# Autodesk Inventor assembly: use this - gimme that tech award
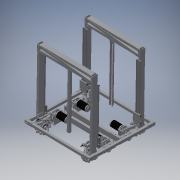
[picture p0: Inventor's stored thumbnail of the model, 180x180]
Saved by Autodesk Inventor 2018 (Build 220112000, 112)
## iProperties
Created: 2019-01-10
Part Number: use this - gimme that tech award
Document SubType Name: Assembly
Designer: maste
Author: maste
## Documents named in this file (6)
- C:\Users\s-2512711\Desktop\Github\2019CAD\Drivebase but Calvin is a mad man\use this - gimme that tech award.iam
- C:\Users\s-2512711\Desktop\Github\2019CAD\Drivebase but Calvin is a mad man\Slidey Mecanum L thing V2.iam
- C:\Users\s-2512711\Desktop\Github\2019CAD\Drivebase but Calvin is a mad man\WW_10_40_10_AL_2.ipt
- C:\Users\s-2512711\Desktop\Github\2019CAD\Drivebase but Calvin is a mad man\91292A197_TYPE 18-8 SS SOCKET HEAD CAP SCREW (1).ipt
- C:\Users\s-2512711\Desktop\Github\2019CAD\Drivebase but Calvin is a mad man\93625A200_TYPE 18-8 STAINLESS STL NYLON-INSERT LOCKNUT.ipt
- C:\Users\s-2512711\Desktop\Github\2019CAD\Drivebase but Calvin is a mad man\Bumper Frame.iam
## Components (23 placed, 5 different names)
1. Slidey Mecanum L thing V2:1 [sub-assembly] — Mate:59, Mate:60, Mate:61, Mate:62, Flush:5, Flush:6, Flush:7, Mate:118
2. Slidey Mecanum L thing V2:2 [sub-assembly] — Mate:55, Mate:56, Mate:57, Mate:58, Flush:3, Flush:4, Mate:115, Mate:116, Mate:117, Flush:7
3. WW_10_40_10_AL_2:1 — Mate:57, Mate:58, Flush:3, Mate:76, Mate:77, Mate:78, Mate:79
4. WW_10_40_10_AL_2:2 — Mate:59, Mate:60, Flush:5, Mate:88, Mate:89, Mate:90, Mate:91
5. WW_10_40_10_AL_2:3 — Mate:61, Mate:62, Flush:6, Mate:84, Mate:85, Mate:86, Mate:87
6. WW_10_40_10_AL_2:4 — Mate:55, Mate:56, Flush:4, Mate:80, Mate:81, Mate:82, Mate:83
7. 91292A197_TYPE 18-8 SS SOCKET HEAD CAP SCREW (1):1 — Mate:76, Mate:77, Mate:106
8. 91292A197_TYPE 18-8 SS SOCKET HEAD CAP SCREW (1):2 — Mate:78, Mate:79, Mate:107
9. 91292A197_TYPE 18-8 SS SOCKET HEAD CAP SCREW (1):3 — Mate:80, Mate:81, Mate:110
10. 91292A197_TYPE 18-8 SS SOCKET HEAD CAP SCREW (1):4 — Mate:82, Mate:83, Mate:111
11. 91292A197_TYPE 18-8 SS SOCKET HEAD CAP SCREW (1):5 — Mate:84, Mate:85, Mate:103
12. 91292A197_TYPE 18-8 SS SOCKET HEAD CAP SCREW (1):6 — Mate:86, Mate:87, Mate:102
13. 91292A197_TYPE 18-8 SS SOCKET HEAD CAP SCREW (1):7 — Mate:90, Mate:91, Mate:99
14. 91292A197_TYPE 18-8 SS SOCKET HEAD CAP SCREW (1):8 — Mate:88, Mate:89, Mate:98
15. 93625A200_TYPE 18-8 STAINLESS STL NYLON-INSERT LOCKNUT:1 — Mate:111
16. 93625A200_TYPE 18-8 STAINLESS STL NYLON-INSERT LOCKNUT:2 — Mate:110
17. 93625A200_TYPE 18-8 STAINLESS STL NYLON-INSERT LOCKNUT:3 — Mate:106
18. 93625A200_TYPE 18-8 STAINLESS STL NYLON-INSERT LOCKNUT:4 — Mate:107
19. 93625A200_TYPE 18-8 STAINLESS STL NYLON-INSERT LOCKNUT:6 — Mate:99
20. 93625A200_TYPE 18-8 STAINLESS STL NYLON-INSERT LOCKNUT:7 — Mate:98
21. 93625A200_TYPE 18-8 STAINLESS STL NYLON-INSERT LOCKNUT:8 — Mate:103
22. 93625A200_TYPE 18-8 STAINLESS STL NYLON-INSERT LOCKNUT:9 — Mate:102
23. Bumper Frame:1 [sub-assembly] — Mate:115, Mate:116, Mate:117, Mate:118
## Relationships (41: Mate 36, Flush 5)
- Mate:55: Slidey Mecanum L thing V2:2 ↔ WW_10_40_10_AL_2:4
- Mate:56: Slidey Mecanum L thing V2:2 ↔ WW_10_40_10_AL_2:4
- Mate:57: Slidey Mecanum L thing V2:2 ↔ WW_10_40_10_AL_2:1
- Mate:58: Slidey Mecanum L thing V2:2 ↔ WW_10_40_10_AL_2:1
- Mate:59: Slidey Mecanum L thing V2:1 ↔ WW_10_40_10_AL_2:2
- Mate:60: Slidey Mecanum L thing V2:1 ↔ WW_10_40_10_AL_2:2
- Mate:61: Slidey Mecanum L thing V2:1 ↔ WW_10_40_10_AL_2:3
- Mate:62: Slidey Mecanum L thing V2:1 ↔ WW_10_40_10_AL_2:3
- Flush:3: Slidey Mecanum L thing V2:2 ↔ WW_10_40_10_AL_2:1
- Flush:4: Slidey Mecanum L thing V2:2 ↔ WW_10_40_10_AL_2:4
- Flush:5: Slidey Mecanum L thing V2:1 ↔ WW_10_40_10_AL_2:2
- Flush:6: Slidey Mecanum L thing V2:1 ↔ WW_10_40_10_AL_2:3
- Mate:76: WW_10_40_10_AL_2:1 ↔ 91292A197_TYPE 18-8 SS SOCKET HEAD CAP SCREW (1):1
- Mate:77: WW_10_40_10_AL_2:1 ↔ 91292A197_TYPE 18-8 SS SOCKET HEAD CAP SCREW (1):1
- Mate:78: WW_10_40_10_AL_2:1 ↔ 91292A197_TYPE 18-8 SS SOCKET HEAD CAP SCREW (1):2
- Mate:79: WW_10_40_10_AL_2:1 ↔ 91292A197_TYPE 18-8 SS SOCKET HEAD CAP SCREW (1):2
- Mate:80: WW_10_40_10_AL_2:4 ↔ 91292A197_TYPE 18-8 SS SOCKET HEAD CAP SCREW (1):3
- Mate:81: WW_10_40_10_AL_2:4 ↔ 91292A197_TYPE 18-8 SS SOCKET HEAD CAP SCREW (1):3
- Mate:82: WW_10_40_10_AL_2:4 ↔ 91292A197_TYPE 18-8 SS SOCKET HEAD CAP SCREW (1):4
- Mate:83: WW_10_40_10_AL_2:4 ↔ 91292A197_TYPE 18-8 SS SOCKET HEAD CAP SCREW (1):4
- Mate:84: WW_10_40_10_AL_2:3 ↔ 91292A197_TYPE 18-8 SS SOCKET HEAD CAP SCREW (1):5
- Mate:85: WW_10_40_10_AL_2:3 ↔ 91292A197_TYPE 18-8 SS SOCKET HEAD CAP SCREW (1):5
- Mate:86: WW_10_40_10_AL_2:3 ↔ 91292A197_TYPE 18-8 SS SOCKET HEAD CAP SCREW (1):6
- Mate:87: WW_10_40_10_AL_2:3 ↔ 91292A197_TYPE 18-8 SS SOCKET HEAD CAP SCREW (1):6
- Mate:88: WW_10_40_10_AL_2:2 ↔ 91292A197_TYPE 18-8 SS SOCKET HEAD CAP SCREW (1):8
- Mate:89: WW_10_40_10_AL_2:2 ↔ 91292A197_TYPE 18-8 SS SOCKET HEAD CAP SCREW (1):8
- Mate:90: WW_10_40_10_AL_2:2 ↔ 91292A197_TYPE 18-8 SS SOCKET HEAD CAP SCREW (1):7
- Mate:91: WW_10_40_10_AL_2:2 ↔ 91292A197_TYPE 18-8 SS SOCKET HEAD CAP SCREW (1):7
- Mate:98: 91292A197_TYPE 18-8 SS SOCKET HEAD CAP SCREW (1):8 ↔ 93625A200_TYPE 18-8 STAINLESS STL NYLON-INSERT LOCKNUT:7
- Mate:99: 91292A197_TYPE 18-8 SS SOCKET HEAD CAP SCREW (1):7 ↔ 93625A200_TYPE 18-8 STAINLESS STL NYLON-INSERT LOCKNUT:6
- Mate:102: 91292A197_TYPE 18-8 SS SOCKET HEAD CAP SCREW (1):6 ↔ 93625A200_TYPE 18-8 STAINLESS STL NYLON-INSERT LOCKNUT:9
- Mate:103: 91292A197_TYPE 18-8 SS SOCKET HEAD CAP SCREW (1):5 ↔ 93625A200_TYPE 18-8 STAINLESS STL NYLON-INSERT LOCKNUT:8
- Mate:106: 91292A197_TYPE 18-8 SS SOCKET HEAD CAP SCREW (1):1 ↔ 93625A200_TYPE 18-8 STAINLESS STL NYLON-INSERT LOCKNUT:3
- Mate:107: 91292A197_TYPE 18-8 SS SOCKET HEAD CAP SCREW (1):2 ↔ 93625A200_TYPE 18-8 STAINLESS STL NYLON-INSERT LOCKNUT:4
- Mate:110: 91292A197_TYPE 18-8 SS SOCKET HEAD CAP SCREW (1):3 ↔ 93625A200_TYPE 18-8 STAINLESS STL NYLON-INSERT LOCKNUT:2
- Mate:111: 91292A197_TYPE 18-8 SS SOCKET HEAD CAP SCREW (1):4 ↔ 93625A200_TYPE 18-8 STAINLESS STL NYLON-INSERT LOCKNUT:1
- Mate:115 (25.4 mm): Slidey Mecanum L thing V2:2 ↔ Bumper Frame:1
- Mate:116: Slidey Mecanum L thing V2:2 ↔ Bumper Frame:1
- Mate:117 (50.8 mm): Slidey Mecanum L thing V2:2 ↔ Bumper Frame:1
- Flush:7: Slidey Mecanum L thing V2:1 ↔ Slidey Mecanum L thing V2:2
- Mate:118 (50.8 mm): Slidey Mecanum L thing V2:1 ↔ Bumper Frame:1
